# Autodesk Inventor assembly: Assembly_sculpt
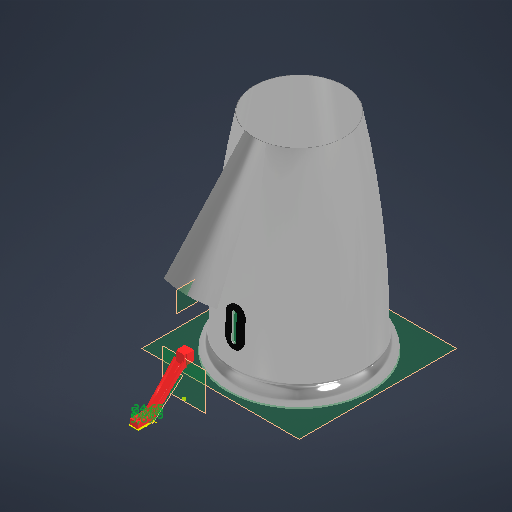
[picture p0: Inventor's stored thumbnail of the model, 512x512]
Saved by Autodesk Inventor 2026 (Build 300175000, 175)
## iProperties
Created: 2025-04-30
Part Number: Assembly_sculpt
Document SubType Name: Assembly
Designer: Paul Juschitz
Author: Paul Juschitz
## Documents named in this file (3)
- C:\Users\Paul Juschitz\Documents\private\m5_GBW_mod\M5_GBW_mod\CAD\Assembly_sculpt.iam
- C:\Users\Paul Juschitz\Documents\private\m5_GBW_mod\M5_GBW_mod\CAD\load_cell_bracket_2.ipt
- C:\Users\Paul Juschitz\Documents\private\m5_GBW_mod\M5_GBW_mod\CAD\m2m_shell_2.ipt
## Components (2 placed, 2 different names)
1. load_cell_bracket_2:1 — Mate:1
2. m2m_shell_2:1 — Mate:1
## Relationships (1: Mate 1)
- Mate:1: load_cell_bracket_2:1 ↔ m2m_shell_2:1
